# Autodesk Inventor assembly: Assembly1
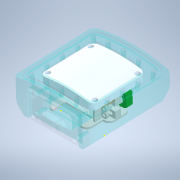
[picture p0: Inventor's stored thumbnail of the model, 180x180]
Saved by Autodesk Inventor 2020 (Build 240168000, 168)
## iProperties
Created: 2019-10-17
Part Number: Assembly1
Document SubType Name: Assembly
Designer: jesse
Author: jesse
## Documents named in this file (11)
- C:\Users\Hymowitz\Documents\Rocksat2020CAD\Port Cover Assembly.iam
- C:\Users\Hymowitz\Documents\Rocksat2020CAD\MultipurposePort-Released_withSTL\Assembly Multipurpose Port.iam
- C:\Users\Hymowitz\Documents\Rocksat2020CAD\camera.ipt
- C:\Users\Hymowitz\Documents\Rocksat2020CAD\s_arm.ipt
- C:\Users\Hymowitz\Documents\Rocksat2020CAD\s_support.ipt
- C:\Users\Hymowitz\Documents\Rocksat2020CAD\MultipurposePort-Released_withSTL\ME112673.ipt
- C:\Users\Hymowitz\Documents\Rocksat2020CAD\adapter_1.ipt
- C:\Users\Hymowitz\Documents\Rocksat2020CAD\s_support_bottom.ipt
- C:\Users\Hymowitz\Documents\Rocksat2020CAD\adapter2.ipt
- C:\Users\Hymowitz\Documents\Rocksat2020CAD\3rd party\micro-metal-gearmotor-1000-backshaft.ipt
- C:\Users\Hymowitz\Documents\Rocksat2020CAD\flatcamera.ipt
## Components (18 placed, 10 different names)
1. Assembly Multipurpose Port:1 [sub-assembly] — Mate:11, Mate:12, Flush:9, Flush:10, Mate:23, Mate:32, Mate:34, Flush:14, Flush:16, Flush:18
2. camera:1 — Mate:13, Flush:5, Flush:6, Flush:7
3. s_arm:1 — Rotational:1, Mate:6, Mate:21
4. s_arm:2 — Rotational:1, Mate:7, Mate:8, Mate:25, Mate:29
5. s_support:3 — Mate:9, Mate:10, Mate:31, Mate:32
6. s_arm:3 — Mate:6, Mate:31
7. s_arm:4 — Mate:7, Mate:8, Mate:9
8. Top Cover — Mate:10, Mate:11, Mate:12, Mate:13, Flush:5, Flush:6, Mate:14, Flush:8, Mate:37, Flush:39
9. camera:2 — Mate:14, Flush:7, Flush:8
10. adapter_1:1 — Flush:9, Flush:10
11. s_arm:5 — Mate:21, Mate:28, Mate:35
12. s_arm:6 — Mate:27
13. s_arm:7 — Mate:38
14. s_arm:8
15. s_support_bottom:1 — Mate:23, Mate:25, Mate:27, Mate:28, Mate:29, Mate:34, Mate:35, Flush:14, Flush:37, Mate:36, Flush:38
16. adapter2:1 — Flush:16, Flush:18
17. micro-metal-gearmotor-1000-backshaft:1 — Flush:37, Mate:36, Flush:38
18. flatcamera:1 — Mate:37, Mate:38, Flush:39
## Relationships (41: Mate 25, Flush 12, RevoluteJoint 4)
- Rotational:1 [RevoluteJoint]: s_arm:1 ↔ s_arm:2
- [RevoluteJoint]: s_arm:3 ↔ s_arm:4
- Mate:6: s_arm:1 ↔ s_arm:3
- Mate:7: s_arm:2 ↔ s_arm:4
- Mate:8: s_arm:2 ↔ s_arm:4
- Mate:9: s_support:3 ↔ s_arm:4
- Mate:10: s_support:3 ↔ Top Cover
- Mate:11: Assembly Multipurpose Port:1 ↔ Top Cover
- Mate:12: Assembly Multipurpose Port:1 ↔ Top Cover
- Mate:13: camera:1 ↔ Top Cover
- Flush:5: camera:1 ↔ Top Cover
- Flush:6 (-29.0068 mm): camera:1 ↔ Top Cover
- Mate:14: Top Cover ↔ camera:2
- Flush:7: camera:1 ↔ camera:2
- Flush:8: Top Cover ↔ camera:2
- Flush:9: Assembly Multipurpose Port:1 ↔ adapter_1:1
- Flush:10: Assembly Multipurpose Port:1 ↔ adapter_1:1
- [RevoluteJoint]: s_arm:5 ↔ s_arm:6
- [RevoluteJoint]: s_arm:7 ↔ s_arm:8
- [Mate]: s_arm:5 ↔ s_arm:7
- [Mate]: s_arm:6 ↔ s_arm:8
- [Mate]: s_arm:6 ↔ s_arm:8
- Mate:21: s_arm:1 ↔ s_arm:5
- Mate:23: Assembly Multipurpose Port:1 ↔ s_support_bottom:1
- Mate:25: s_arm:2 ↔ s_support_bottom:1
- Mate:27: s_arm:6 ↔ s_support_bottom:1
- Mate:28: s_arm:5 ↔ s_support_bottom:1
- Mate:29: s_arm:2 ↔ s_support_bottom:1
- Mate:31: s_support:3 ↔ s_arm:3
- Mate:32: Assembly Multipurpose Port:1 ↔ s_support:3
- Mate:34 (26.21 mm): Assembly Multipurpose Port:1 ↔ s_support_bottom:1
- Mate:35: s_arm:5 ↔ s_support_bottom:1
- Flush:14: Assembly Multipurpose Port:1 ↔ s_support_bottom:1
- Flush:16: Assembly Multipurpose Port:1 ↔ adapter2:1
- Flush:18: Assembly Multipurpose Port:1 ↔ adapter2:1
- Flush:37: s_support_bottom:1 ↔ micro-metal-gearmotor-1000-backshaft:1
- Mate:36: s_support_bottom:1 ↔ micro-metal-gearmotor-1000-backshaft:1
- Flush:38: s_support_bottom:1 ↔ micro-metal-gearmotor-1000-backshaft:1
- Mate:37: Top Cover ↔ flatcamera:1
- Mate:38: s_arm:7 ↔ flatcamera:1
- Flush:39: Top Cover ↔ flatcamera:1
## Named parameters: support_length = 58.42 mm, s_arm_length = 58.42 mm, d17_d2 = 0 mm, d18_d3 = 164.577708 deg, d41_d2 = 0 mm, d42_d3 = -15.422292 deg, d43_d17_d2 = 0 mm, d44_d18_d3 = 164.577708 deg, d45_d21 = 0 mm, d46_d22 = 0 mm, d47_d23 = 0 mm
